# Autodesk Inventor assembly: Wood_X_Frame
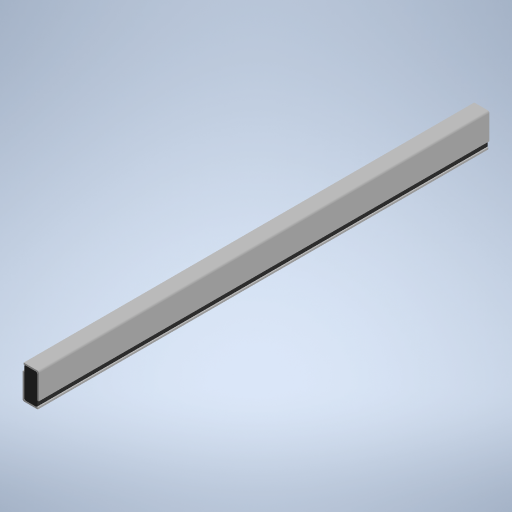
[picture p0: Inventor's stored thumbnail of the model, 512x512]
Saved by Autodesk Inventor 2023 (Build 270158000, 158)
## iProperties
Created: 2022-05-10
Part Number: Wood_X_Frame
Document SubType Name: Assembly
Designer: a laptop
Author: a laptop
## Documents named in this file (13)
- D:\Users\plebbb\Desktop\CNC_Project\Wood_X_Frame.iam
- D:\Users\plebbb\Desktop\CNC_Project\L_Channel.ipt
- D:\Users\plebbb\Desktop\CNC_Project\2x4_Wood.ipt
- D:\Users\plebbb\Desktop\CNC_Project\Wood_X_Frame\AIP\FEA\dytmg7jgg.fins
- D:\Users\plebbb\Desktop\CNC_Project\Wood_X_Frame\AIP\FEA\dytmg7jgg.fsat
- D:\Users\plebbb\Desktop\CNC_Project\Wood_X_Frame\AIP\FEA\dytmg7jhc.ftes
- D:\Users\plebbb\Desktop\CNC_Project\Wood_X_Frame\AIP\FEA\dytmg7jhc.fwiz
- D:\Users\plebbb\Desktop\CNC_Project\Wood_X_Frame\AIP\FEA\dytmg7jkw.fmsh
- D:\Users\plebbb\Desktop\CNC_Project\Wood_X_Frame\AIP\FEA\dytmg7jkx.fres
- D:\Users\plebbb\Desktop\CNC_Project\Wood_X_Frame\AIP\FEA\dytmg7jpc.fmsh
- D:\Users\plebbb\Desktop\CNC_Project\Wood_X_Frame\AIP\FEA\dytmg7jq8.fres
- D:\Users\plebbb\Desktop\CNC_Project\Wood_X_Frame\AIP\FEA\dytxt4xi8.fmsh
- D:\Users\plebbb\Desktop\CNC_Project\Wood_X_Frame\AIP\FEA\dytxt4xi9.fres
## Components (3 placed, 2 different names)
1. L_Channel:1
2. 2x4_Wood:1
3. L_Channel:2
## Relationships (6: Mate 4, Flush 2)
- [Mate]: L_Channel:1 ↔ 2x4_Wood:1
- [Mate]: L_Channel:1 ↔ 2x4_Wood:1
- [Flush]: L_Channel:1 ↔ 2x4_Wood:1
- [Flush]: 2x4_Wood:1 ↔ L_Channel:2
- [Mate]: 2x4_Wood:1 ↔ L_Channel:2
- [Mate]: 2x4_Wood:1 ↔ L_Channel:2
## Named parameters: sa_1 = 58800, sa_0 = 100000, sa_2 = 100000
note: some values were not read from the file. Shown as the stored number, unit unknown: "sa_1", "sa_0", "sa_2".
